# Autodesk Inventor assembly: Mauro_Wagen_QR_version
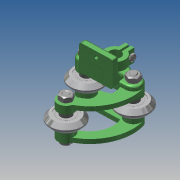
[picture p0: Inventor's stored thumbnail of the model, 180x180]
Saved by Autodesk Inventor 2015 SP1 (Build 190203100, 203)
## iProperties
Created: 2015-03-04
Part Number: Mauro_Wagen_QR_version
Document SubType Name: Assembly
Designer: Marc
Author: Marc
## Documents named in this file (9)
- E:\Modellflieger\3D Drucker\Eigene Teile\LinearWagen_Mauro_Wheels\Mauro_Wagen_QR_version.iam
- E:\Modellflieger\3D Drucker\Eigene Teile\LinearWagen_Mauro_Wheels\Linearwagen_MauroW_inside.ipt
- E:\Modellflieger\3D Drucker\Eigene Teile\LinearWagen_Mauro_Wheels\Mauro_White_Wheel.ipt
- C:\Users\Marc\Documents\Inventor\Content Center Files\R2015\de-DE\DIN 84\DIN 84 - M6 x 40.ipt
- C:\Users\Marc\Documents\Inventor\Content Center Files\R2015\de-DE\DIN 84\DIN 84 - M6 x 35.ipt
- C:\Users\Marc\Documents\Inventor\Content Center Files\R2015\de-DE\DIN 934\DIN 934 - M6 x 1.ipt
- C:\Users\Marc\Documents\Inventor\Content Center Files\R2015\de-DE\DIN 84\DIN 84 - M3 x 10.ipt
- C:\Users\Marc\Documents\Inventor\Content Center Files\R2015\de-DE\DIN 934\DIN 934 - M3 x 0,5.ipt
- E:\Modellflieger\3D Drucker\Eigene Teile\LinearWagen_Mauro_Wheels\Linearwagen_MauroW_outside_QR-version.ipt
## Components (13 placed, 8 different names)
1. Linearwagen_MauroW_inside:1 — Einfügen:4, Einfügen:5, Einfügen:6, Einfügen:7, Einfügen:8
2. Linearwagen_MauroW_outside_QR-version:1 — Einfügen:1, Einfügen:2, Einfügen:3, Passend:2, Passend:4, Passend:6, Einfügen:9, Passend:8
3. Mauro_White_Wheel:1 — Einfügen:1, Einfügen:4
4. Mauro_White_Wheel:2 — Einfügen:3
5. Mauro_White_Wheel:3 — Einfügen:2, Einfügen:5
6. DIN 84 - ersetzt durch DIN EN ISO 1207 M6 x 40:1 — Einfügen:7, Passend:3
7. DIN 84 - ersetzt durch DIN EN ISO 1207 M6 x 40:2 — Einfügen:6, Passend:1
8. DIN 84 - ersetzt durch DIN EN ISO 1207 M6 x 35:1 — Einfügen:8, Passend:5
9. DIN 934 - ersetzt durch DIN EN 24032/28673/28674 M6:1 — Passend:1, Passend:2
10. DIN 934 - ersetzt durch DIN EN 24032/28673/28674 M6:2 — Passend:3, Passend:4
11. DIN 934 - ersetzt durch DIN EN 24032/28673/28674 M6:3 — Passend:5, Passend:6
12. DIN 84 - ersetzt durch DIN EN ISO 1207 M3 x 10:1 — Einfügen:9, Passend:7
13. DIN 934 - ersetzt durch DIN EN 24032/28673/28674 M3:1 — Passend:7, Passend:8
## Relationships (17: Insert 9, Mate 8)
- Einfügen:1 [Insert]: Linearwagen_MauroW_outside_QR-version:1 ↔ Mauro_White_Wheel:1
- Einfügen:2 [Insert]: Linearwagen_MauroW_outside_QR-version:1 ↔ Mauro_White_Wheel:3
- Einfügen:3 [Insert]: Linearwagen_MauroW_outside_QR-version:1 ↔ Mauro_White_Wheel:2
- Einfügen:4 [Insert]: Linearwagen_MauroW_inside:1 ↔ Mauro_White_Wheel:1
- Einfügen:5 [Insert]: Linearwagen_MauroW_inside:1 ↔ Mauro_White_Wheel:3
- Einfügen:6 [Insert]: Linearwagen_MauroW_inside:1 ↔ DIN 84 - ersetzt durch DIN EN ISO 1207 M6 x 40:2
- Einfügen:7 [Insert]: Linearwagen_MauroW_inside:1 ↔ DIN 84 - ersetzt durch DIN EN ISO 1207 M6 x 40:1
- Einfügen:8 [Insert]: Linearwagen_MauroW_inside:1 ↔ DIN 84 - ersetzt durch DIN EN ISO 1207 M6 x 35:1
- Passend:1 [Mate]: DIN 84 - ersetzt durch DIN EN ISO 1207 M6 x 40:2 ↔ DIN 934 - ersetzt durch DIN EN 24032/28673/28674 M6:1
- Passend:2 [Mate]: Linearwagen_MauroW_outside_QR-version:1 ↔ DIN 934 - ersetzt durch DIN EN 24032/28673/28674 M6:1
- Passend:3 [Mate]: DIN 84 - ersetzt durch DIN EN ISO 1207 M6 x 40:1 ↔ DIN 934 - ersetzt durch DIN EN 24032/28673/28674 M6:2
- Passend:4 [Mate]: Linearwagen_MauroW_outside_QR-version:1 ↔ DIN 934 - ersetzt durch DIN EN 24032/28673/28674 M6:2
- Passend:5 [Mate]: DIN 84 - ersetzt durch DIN EN ISO 1207 M6 x 35:1 ↔ DIN 934 - ersetzt durch DIN EN 24032/28673/28674 M6:3
- Passend:6 [Mate]: Linearwagen_MauroW_outside_QR-version:1 ↔ DIN 934 - ersetzt durch DIN EN 24032/28673/28674 M6:3
- Einfügen:9 [Insert]: Linearwagen_MauroW_outside_QR-version:1 ↔ DIN 84 - ersetzt durch DIN EN ISO 1207 M3 x 10:1
- Passend:7 [Mate]: DIN 84 - ersetzt durch DIN EN ISO 1207 M3 x 10:1 ↔ DIN 934 - ersetzt durch DIN EN 24032/28673/28674 M3:1
- Passend:8 [Mate]: Linearwagen_MauroW_outside_QR-version:1 ↔ DIN 934 - ersetzt durch DIN EN 24032/28673/28674 M3:1
